# Autodesk Inventor assembly: Assembly13
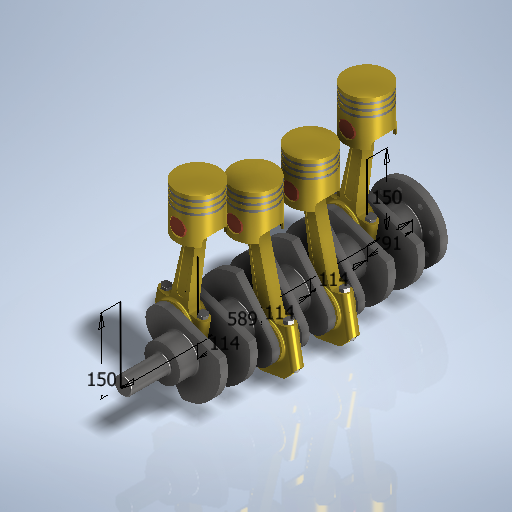
[picture p0: Inventor's stored thumbnail of the model, 512x512]
Saved by Autodesk Inventor 2025.2 (Build 292293000, 293)
## iProperties
Created: 2025-03-20
Part Number: Assembly13
Document SubType Name: Assembly
Designer: User
Author: User
## Documents named in this file (5)
- C:\Users\User\Documents\Inventor\Engine\Assembly13.iam
- C:\Users\User\Documents\Inventor\Engine\Part 2 Crankshaft.ipt
- C:\Users\User\Documents\Inventor\Engine\Sketch.ipt
- C:\Users\User\Documents\Inventor\Engine\A.iam
- C:\Users\User\Documents\Inventor\Engine\B.iam
## Components (10 placed, 4 different names)
1. Part 2 Crankshaft:1 — Mate:1, Flush:1, Mate:6, Mate:7, Mate:8, Mate:9, Mate:10, Mate:11, Mate:12, Mate:13
2. Sketch:1 — Mate:1, Flush:1, Mate:2, Mate:3, Mate:4, Mate:5
3. A:1 [sub-assembly] — Mate:2, Mate:14
4. A:2 [sub-assembly] — Mate:3, Mate:15
5. A:3 [sub-assembly] — Mate:4, Mate:16
6. A:4 [sub-assembly] — Mate:5, Mate:17
7. B:1 [sub-assembly] — Mate:12, Mate:13, Mate:17
8. B:2 [sub-assembly] — Mate:6, Mate:7, Mate:14
9. B:3 [sub-assembly] — Mate:8, Mate:9, Mate:15
10. B:4 [sub-assembly] — Mate:10, Mate:11, Mate:16
## Relationships (18: Mate 17, Flush 1)
- Mate:1: Part 2 Crankshaft:1 ↔ Sketch:1
- Flush:1: Part 2 Crankshaft:1 ↔ Sketch:1
- Mate:2: Sketch:1 ↔ A:1
- Mate:3: Sketch:1 ↔ A:2
- Mate:4: Sketch:1 ↔ A:3
- Mate:5: Sketch:1 ↔ A:4
- Mate:6: Part 2 Crankshaft:1 ↔ B:2
- Mate:7 (3.5 mm): Part 2 Crankshaft:1 ↔ B:2
- Mate:8: Part 2 Crankshaft:1 ↔ B:3
- Mate:9 (3.4 mm): Part 2 Crankshaft:1 ↔ B:3
- Mate:10: Part 2 Crankshaft:1 ↔ B:4
- Mate:11 (3.4 mm): Part 2 Crankshaft:1 ↔ B:4
- Mate:12: Part 2 Crankshaft:1 ↔ B:1
- Mate:13 (3.4 mm): Part 2 Crankshaft:1 ↔ B:1
- Mate:14: A:1 ↔ B:2
- Mate:15: A:2 ↔ B:3
- Mate:16: A:3 ↔ B:4
- Mate:17: A:4 ↔ B:1
